# Autodesk Inventor assembly: tssopСборка
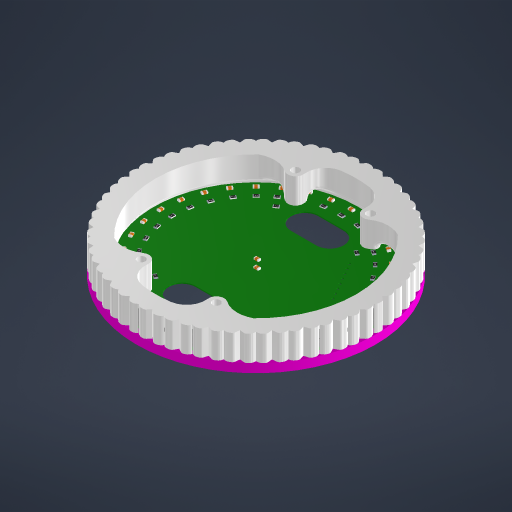
[picture p0: Inventor's stored thumbnail of the model, 512x512]
Saved by Autodesk Inventor 2023 (Build 270158000, 158)
## iProperties
Created: 2025-01-12
Part Number: tssopСборка
Document SubType Name: Assembly
Designer: Ivan
Mass: 37.2912 g
Surface Area: 543.372 cm^2
Volume: 37.2912 cm^3
Density: 1 g/cm^3
Author: Ivan
## Documents named in this file (8)
- C:\!projects\dash_localDirectory\DASH_\Dash-V1\step\tssp\tssopСборка.iam
- C:\!projects\dash_localDirectory\DASH_\Dash-V1\tssop3D\tssop3D (3).iam
- C:\!projects\dash_localDirectory\DASH_\Dash-V1\step\tssp\User Library-TSSP40_IR reciver.ipt
- C:\!projects\dash_localDirectory\DASH_\Dash-V1\tsspLid2.ipt
- C:\!projects\dash_localDirectory\DASH_\Dash-V1\step\tssp\tssopLid3.ipt
- C:\!projects\dash_localDirectory\DASH_\Dash-V1\Dribler\DriblerPlatform.ipt
- C:\!projects\dash_localDirectory\DASH_\Dash-V1\step\tssp\tssopLid3.1.ipt
- C:\!projects\dash_localDirectory\DASH_\Dash-V1\step\tssp\кольцо тсопов.ipt
## Components (38 placed, 7 different names)
1. tssop3D (3):1 [sub-assembly] — Совмещение:1, Совмещение:2, Совмещение:3, Совмещение:4, Совмещение:5, Угол:1, Заподлицо:1, Заподлицо:2, Заподлицо:3, Заподлицо:4, Совмещение:8
2. tsspLid2:1 — Заподлицо:1, Заподлицо:2
3. tssopLid3:1 — Заподлицо:3, Заподлицо:4, Совмещение:6, Совмещение:7
4. DriblerPlatform:1 — Совмещение:6, Совмещение:7
5. tssopLid3.1:1 — Совмещение:8, Заподлицо:5, Заподлицо:6
6. кольцо тсопов:1 — Заподлицо:5, Заподлицо:6
7. User Library-TSSP40_IR reciver:1 — Совмещение:3, Совмещение:4, Совмещение:5
8. User Library-TSSP40_IR reciver:2
9. User Library-TSSP40_IR reciver:3
10. User Library-TSSP40_IR reciver:4
11. User Library-TSSP40_IR reciver:5
12. User Library-TSSP40_IR reciver:6
13. User Library-TSSP40_IR reciver:7
14. User Library-TSSP40_IR reciver:8
15. User Library-TSSP40_IR reciver:9
16. User Library-TSSP40_IR reciver:10
17. User Library-TSSP40_IR reciver:11
18. User Library-TSSP40_IR reciver:12
19. User Library-TSSP40_IR reciver:13
20. User Library-TSSP40_IR reciver:14
21. User Library-TSSP40_IR reciver:15
22. User Library-TSSP40_IR reciver:16
23. User Library-TSSP40_IR reciver:17
24. User Library-TSSP40_IR reciver:18
25. User Library-TSSP40_IR reciver:19
26. User Library-TSSP40_IR reciver:20
27. User Library-TSSP40_IR reciver:21
28. User Library-TSSP40_IR reciver:22
29. User Library-TSSP40_IR reciver:23
30. User Library-TSSP40_IR reciver:24
31. User Library-TSSP40_IR reciver:25
32. User Library-TSSP40_IR reciver:26
33. User Library-TSSP40_IR reciver:27
34. User Library-TSSP40_IR reciver:28
35. User Library-TSSP40_IR reciver:29
36. User Library-TSSP40_IR reciver:30
37. User Library-TSSP40_IR reciver:31
38. User Library-TSSP40_IR reciver:32
## Component patterns: (32 elements, first: User Library-TSSP40_IR reciver:1)
## Relationships (15: Mate 8, Flush 6, Angle 1)
- Совмещение:1 [Mate]: tssop3D (3):1
- Совмещение:2 [Mate]: tssop3D (3):1
- Совмещение:3 [Mate]: tssop3D (3):1 ↔ User Library-TSSP40_IR reciver:1
- Совмещение:4 [Mate]: tssop3D (3):1 ↔ User Library-TSSP40_IR reciver:1
- Совмещение:5 [Mate]: tssop3D (3):1 ↔ User Library-TSSP40_IR reciver:1
- Угол:1 [Angle] (0 deg): tssop3D (3):1
- Заподлицо:1 [Flush]: tssop3D (3):1 ↔ tsspLid2:1
- Заподлицо:2 [Flush]: tssop3D (3):1 ↔ tsspLid2:1
- Заподлицо:3 [Flush]: tssop3D (3):1 ↔ tssopLid3:1
- Заподлицо:4 [Flush]: tssop3D (3):1 ↔ tssopLid3:1
- Совмещение:6 [Mate]: tssopLid3:1 ↔ DriblerPlatform:1
- Совмещение:7 [Mate]: tssopLid3:1 ↔ DriblerPlatform:1
- Совмещение:8 [Mate]: tssop3D (3):1 ↔ tssopLid3.1:1
- Заподлицо:5 [Flush]: tssopLid3.1:1 ↔ кольцо тсопов:1
- Заподлицо:6 [Flush]: tssopLid3.1:1 ↔ кольцо тсопов:1
